# Autodesk Inventor assembly: TerminalBlock
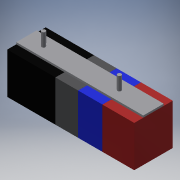
[picture p0: Inventor's stored thumbnail of the model, 180x180]
Saved by Autodesk Inventor 2017 (Build 210142000, 142)
## iProperties
Created: 2017-02-10
Part Number: TerminalBlock
Document SubType Name: Assembly
Designer: michael
Author: michael
## Documents named in this file (6)
- C:\Users\michael\Documents\Jinx\Parts\TerminalBlock.iam
- C:\Users\michael\Documents\Jinx\Parts\Gnd_Terminal.ipt
- C:\Users\michael\Documents\Jinx\Parts\5vTerminal.ipt
- C:\Users\michael\Documents\Jinx\Parts\12vTerminal.ipt
- C:\Users\michael\Documents\Jinx\Parts\24vTerminal.ipt
- C:\Users\michael\Documents\Jinx\Parts\DinRail.ipt
## Components (5 placed, 5 different names)
1. Gnd_Terminal:1 — Mate:1, Mate:2, Mate:3
2. 5vTerminal:1 — Mate:1, Mate:2, Mate:3, Mate:4, Mate:5, Mate:6
3. 12vTerminal:1 — Mate:4, Mate:5, Mate:6, Mate:7, Mate:8, Mate:9, Mate:12
4. 24vTerminal:1 — Mate:7, Mate:8, Mate:9, Mate:10, Mate:11
5. DinRail:1 — Mate:10, Mate:11, Mate:12
## Relationships (12: Mate 12)
- Mate:1: Gnd_Terminal:1 ↔ 5vTerminal:1
- Mate:2: Gnd_Terminal:1 ↔ 5vTerminal:1
- Mate:3: Gnd_Terminal:1 ↔ 5vTerminal:1
- Mate:4: 5vTerminal:1 ↔ 12vTerminal:1
- Mate:5: 5vTerminal:1 ↔ 12vTerminal:1
- Mate:6: 5vTerminal:1 ↔ 12vTerminal:1
- Mate:7: 12vTerminal:1 ↔ 24vTerminal:1
- Mate:8: 12vTerminal:1 ↔ 24vTerminal:1
- Mate:9: 12vTerminal:1 ↔ 24vTerminal:1
- Mate:10: 24vTerminal:1 ↔ DinRail:1
- Mate:11: 24vTerminal:1 ↔ DinRail:1
- Mate:12 (11.8999 mm): 12vTerminal:1 ↔ DinRail:1
